# Autodesk Inventor assembly: Edges Assembly
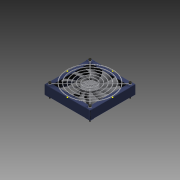
[picture p0: Inventor's stored thumbnail of the model, 180x180]
Saved by Autodesk Inventor 2016 (Build 200138000, 138)
## iProperties
Created: 2015-10-19
Part Number: Edges Assembly
Document SubType Name: Assembly
Designer: Rus
Author: Rus
## Documents named in this file (5)
- C:\Users\Rus\Desktop\AnywhereFan\Edges Assembly.iam
- C:\Users\Rus\Desktop\AnywhereFan\Fractal Design Silent Series R2 140mm.iam
- C:\Users\Rus\Desktop\AnywhereFan\Edge.ipt
- C:\Users\Rus\Desktop\AnywhereFan\Grill.ipt
- C:\Users\Rus\Desktop\AnywhereFan\Screws.ipt
## Components (10 placed, 4 different names)
1. Fractal Design Silent Series R2 140mm:1 [sub-assembly] — Tangent:5, Tangent:6, Tangent:7, Mate:2, Tangent:8, Tangent:9, Tangent:10, Tangent:11, Mate:4, Tangent:20, Mate:7, Mate:10
2. Edge:1 — Flush:1, Mate:1, Tangent:1, Tangent:2, Angle:2, Angle:3, Tangent:21, Insert:1
3. Edge:2 — Flush:2, Flush:3, Tangent:3, Tangent:4, Mate:2, Tangent:9, Angle:1, Angle:4, Mate:6, Tangent:24
4. Edge:3 — Flush:1, Flush:2, Mate:1, Tangent:1, Tangent:4, Tangent:5, Tangent:7, Angle:2, Angle:4, Tangent:22
5. Edge:4 — Flush:3, Tangent:2, Tangent:3, Tangent:6, Tangent:8, Tangent:10, Tangent:11, Angle:1, Angle:3, Angle:5, Angle:8, Tangent:23
6. Grill:1 — Angle:7, Mate:8, Mate:11, Tangent:21
7. Screws:1 — Flush:4, Insert:1
8. Screws:2 — Flush:5, Tangent:22
9. Screws:3 — Flush:5, Flush:6, Tangent:24
10. Screws:4 — Flush:4, Flush:6, Tangent:23
## Relationships (40: Tangent 16, Mate 10, Angle 7, Flush 6, Insert 1)
- Flush:1: Edge:1 ↔ Edge:3
- Flush:2: Edge:2 ↔ Edge:3
- Flush:3: Edge:2 ↔ Edge:4
- Mate:1 (0.0625 mm): Edge:1 ↔ Edge:3
- Tangent:1: Edge:1 ↔ Edge:3
- Tangent:2: Edge:1 ↔ Edge:4
- Tangent:3: Edge:2 ↔ Edge:4
- Tangent:4: Edge:2 ↔ Edge:3
- Tangent:5: Fractal Design Silent Series R2 140mm:1 ↔ Edge:3
- Tangent:6: Fractal Design Silent Series R2 140mm:1 ↔ Edge:4
- Tangent:7: Fractal Design Silent Series R2 140mm:1 ↔ Edge:3
- Mate:2 (1 mm): Fractal Design Silent Series R2 140mm:1 ↔ Edge:2
- Tangent:8: Fractal Design Silent Series R2 140mm:1 ↔ Edge:4
- Tangent:9: Fractal Design Silent Series R2 140mm:1 ↔ Edge:2
- Tangent:10: Fractal Design Silent Series R2 140mm:1 ↔ Edge:4
- Tangent:11: Fractal Design Silent Series R2 140mm:1 ↔ Edge:4
- Angle:1 (90 deg): Edge:2 ↔ Edge:4
- Angle:2 (90 deg): Edge:1 ↔ Edge:3
- Angle:3 (90 deg): Edge:1 ↔ Edge:4
- Angle:4 (90 deg): Edge:2 ↔ Edge:3
- Mate:4: Fractal Design Silent Series R2 140mm:1
- Tangent:20 (2.2 mm): Fractal Design Silent Series R2 140mm:1
- Mate:6: Edge:2
- Angle:5 (0 deg): Edge:4
- Angle:7 (0 deg): Grill:1
- Angle:8 (0 deg): Edge:4
- Mate:7: Fractal Design Silent Series R2 140mm:1
- Mate:8: Grill:1
- Mate:9
- Mate:10: Fractal Design Silent Series R2 140mm:1
- Mate:11: Grill:1
- Mate:12
- Tangent:21: Edge:1 ↔ Grill:1
- Flush:4: Screws:1 ↔ Screws:4
- Flush:5: Screws:2 ↔ Screws:3
- Flush:6: Screws:3 ↔ Screws:4
- Insert:1 (2 mm): Edge:1 ↔ Screws:1
- Tangent:22: Edge:3 ↔ Screws:2
- Tangent:23: Edge:4 ↔ Screws:4
- Tangent:24: Edge:2 ↔ Screws:3
